# Autodesk Inventor assembly: USB
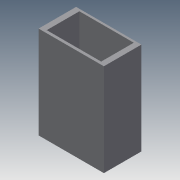
[picture p0: Inventor's stored thumbnail of the model, 180x180]
Saved by Autodesk Inventor 2019 (Build 230136000, 136)
## iProperties
Created: 2019-06-02
Part Number: USB
Document SubType Name: Assembly
Designer: giacomo
Author: giacomo
## Documents named in this file (2)
- D:\Hobby\Inventor\Case 3Dprinted\Prove\USB.iam
- D:\Hobby\Inventor\Case 3Dprinted\B\Case_B2.ipt
## Components (1 placed, 1 different names)
1. Case_B2:1 — Flush:2, Flush:4, Flush:5, Flush:6, Flush:7
## Relationships (5: Flush 5)
- Flush:2: Case_B2:1
- Flush:4 (-1 mm): Case_B2:1
- Flush:5: Case_B2:1
- Flush:6: Case_B2:1
- Flush:7: Case_B2:1
